# Autodesk Inventor assembly: coupler extenison arm motor+ servo mount
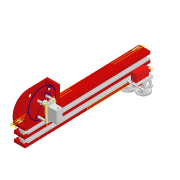
[picture p0: Inventor's stored thumbnail of the model, 180x180]
Saved by Autodesk Inventor 2020 (Build 240168000, 168)
## iProperties
Created: 2019-12-15
Part Number: coupler extenison arm motor+ servo mount
Document SubType Name: Assembly
Designer: ball
Author: ball
## Documents named in this file (14)
- C:\FTC\FTC8863CAD\2019 Robot\Delivery\extension arm\coupler extenison arm motor+ servo mount.iam
- C:\FTC\FTC8863CAD\2019 Robot\Delivery\extension arm\Coupler extension arm motor.ipt
- C:\FTC\FTC8863CAD\2019 Robot\Delivery\extension arm\whole servo mount.ipt
- C:\FTC\FTC8863CAD\2019 Robot\Delivery\extension arm\servo.iam
- C:\FTC\FTC8863CAD\2019 Robot\Delivery\extension arm\Coupler extension arm short.ipt
- C:\FTC\FTC8863CAD\Misumi\SAR340\SAR340 offset 10 mm.iam
- C:\FTC\FTC8863CAD\RevRobotics\REV-41-1368 pulley.ipt
- C:\FTC\FTC8863CAD\2019 Robot\Delivery\plastic pulley deep u.ipt
- C:\FTC\FTC8863CAD\2019 Robot\Delivery\extension arm\extension arm top.iam
- C:\FTC\FTC8863CAD\2019 Robot\Collection\servo block assembly.iam
- C:\FTC\FTC8863CAD\2019 Robot\Delivery\extension arm\Coupler extension arm short edited holes for servo.ipt
- C:\FTC\FTC8863CAD\Actobotics\615 parts\615190.ipt
- C:\FTC\FTC8863CAD\Actobotics\545 parts\545364 assembly.ipt
- C:\FTC\FTC8863CAD\2019 Robot\Delivery\extension arm\standoff for gripper servo.ipt
## Components (18 placed, 13 different names)
1. Coupler extension arm motor:1 — Flush:1, Flush:2, Flush:3, Angle:1, Mate:3, Flush:4, Flush:5, Flush:6, Flush:7, Mate:5, Mate:6, Mate:7, Flush:8, Flush:10, Flush:11
2. whole servo mount:1 — Flush:1, Flush:2, Flush:3, Mate:1, Mate:2
3. servo:1 [sub-assembly] — Mate:1, Mate:2, Angle:1
4. Coupler extension arm short:1 — Mate:3, Flush:4, Flush:5, Mate:4, Mate:8, Mate:9, Mate:10, Mate:11, Mate:12, Flush:9
5. SAR340 offset 10 mm:1 [sub-assembly] — Mate:4, Flush:6, Flush:7, Mate:13
6. REV-41-1368 pulley:1 — Mate:5, Mate:6
7. REV-41-1368 pulley:2 — Mate:7, Flush:8
8. REV-41-1368 pulley:3 — Mate:9, Mate:10
9. REV-41-1368 pulley:4 — Mate:8, Mate:11
10. plastic pulley deep u:1 — Mate:12, Flush:9
11. extension arm top:1 [sub-assembly] — Mate:13, Flush:10, Flush:11, Mate:15, Flush:14, Flush:15
12. Coupler extension arm motor:2 — Flush:12, Flush:13, Mate:14, Mate:15, Flush:14, Flush:15
13. Coupler extension arm short edited holes for servo:1 — Flush:12, Flush:13, Mate:14, Mate:16, Mate:17, Mate:25, Mate:26, Mate:27
14. servo block assembly:1 [sub-assembly] — Mate:16, Mate:17, Mate:19, Mate:22, Mate:28
15. 615190:1 — Mate:19, Flush:16, Mate:21, Mate:23, Mate:24
16. 615190:2 — Flush:16, Mate:21, Mate:22
17. 545364 assembly:1 — Mate:23, Mate:24
18. standoff for gripper servo:1 — Mate:25, Mate:26, Mate:27, Mate:28
## Relationships (43: Mate 26, Flush 16, Angle 1)
- Flush:1: Coupler extension arm motor:1 ↔ whole servo mount:1
- Flush:2: Coupler extension arm motor:1 ↔ whole servo mount:1
- Flush:3: Coupler extension arm motor:1 ↔ whole servo mount:1
- Mate:1: whole servo mount:1 ↔ servo:1
- Mate:2: whole servo mount:1 ↔ servo:1
- Angle:1 (0 deg): Coupler extension arm motor:1 ↔ servo:1
- Mate:3: Coupler extension arm motor:1 ↔ Coupler extension arm short:1
- Flush:4: Coupler extension arm motor:1 ↔ Coupler extension arm short:1
- Flush:5: Coupler extension arm motor:1 ↔ Coupler extension arm short:1
- Mate:4: Coupler extension arm short:1 ↔ SAR340 offset 10 mm:1
- Flush:6: Coupler extension arm motor:1 ↔ SAR340 offset 10 mm:1
- Flush:7: Coupler extension arm motor:1 ↔ SAR340 offset 10 mm:1
- Mate:5: Coupler extension arm motor:1 ↔ REV-41-1368 pulley:1
- Mate:6: Coupler extension arm motor:1 ↔ REV-41-1368 pulley:1
- Mate:7: Coupler extension arm motor:1 ↔ REV-41-1368 pulley:2
- Flush:8: Coupler extension arm motor:1 ↔ REV-41-1368 pulley:2
- Mate:8: Coupler extension arm short:1 ↔ REV-41-1368 pulley:4
- Mate:9: Coupler extension arm short:1 ↔ REV-41-1368 pulley:3
- Mate:10: Coupler extension arm short:1 ↔ REV-41-1368 pulley:3
- Mate:11: Coupler extension arm short:1 ↔ REV-41-1368 pulley:4
- Mate:12: Coupler extension arm short:1 ↔ plastic pulley deep u:1
- Flush:9: Coupler extension arm short:1 ↔ plastic pulley deep u:1
- Mate:13: SAR340 offset 10 mm:1 ↔ extension arm top:1
- Flush:10: Coupler extension arm motor:1 ↔ extension arm top:1
- Flush:11: Coupler extension arm motor:1 ↔ extension arm top:1
- Flush:12: Coupler extension arm motor:2 ↔ Coupler extension arm short edited holes for servo:1
- Flush:13: Coupler extension arm motor:2 ↔ Coupler extension arm short edited holes for servo:1
- Mate:14: Coupler extension arm motor:2 ↔ Coupler extension arm short edited holes for servo:1
- Mate:15: extension arm top:1 ↔ Coupler extension arm motor:2
- Flush:14: extension arm top:1 ↔ Coupler extension arm motor:2
- Flush:15: extension arm top:1 ↔ Coupler extension arm motor:2
- Mate:16: Coupler extension arm short edited holes for servo:1 ↔ servo block assembly:1
- Mate:17: Coupler extension arm short edited holes for servo:1 ↔ servo block assembly:1
- Mate:19: servo block assembly:1 ↔ 615190:1
- Flush:16: 615190:1 ↔ 615190:2
- Mate:21 (38.1 mm): 615190:1 ↔ 615190:2
- Mate:22: servo block assembly:1 ↔ 615190:2
- Mate:23: 615190:1 ↔ 545364 assembly:1
- Mate:24: 615190:1 ↔ 545364 assembly:1
- Mate:25: Coupler extension arm short edited holes for servo:1 ↔ standoff for gripper servo:1
- Mate:26: Coupler extension arm short edited holes for servo:1 ↔ standoff for gripper servo:1
- Mate:27: Coupler extension arm short edited holes for servo:1 ↔ standoff for gripper servo:1
- Mate:28: servo block assembly:1 ↔ standoff for gripper servo:1
